# Autodesk Inventor assembly: HW2_1_task1_var4
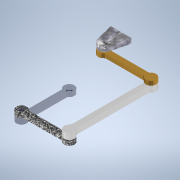
[picture p0: Inventor's stored thumbnail of the model, 180x180]
Saved by Autodesk Inventor 2022 (Build 260153000, 153)
## iProperties
Created: 2022-01-27
Part Number: HW2_1_task1_var4
Document SubType Name: Assembly
Designer: Administrator
Title: HW2_1_task1_var4 v1
Author: Administrator
## Documents named in this file (5)
- C:\Users\br4ch\M-and-Ms\HW2\Task3\Inventor\HW2_1_task1_var4.iam
- C:\Users\br4ch\M-and-Ms\HW2\Task3\Inventor\Machovik_Dlinn.ipt
- C:\Users\br4ch\M-and-Ms\HW2\Task3\Inventor\machovik_2_durki.ipt
- C:\Users\br4ch\M-and-Ms\HW2\Task3\Inventor\machovik.ipt
- C:\Users\br4ch\M-and-Ms\HW2\Task3\Inventor\kronsht.ipt
## Components (5 placed, 4 different names)
1. Machovik_Dlinn:1 — Cylindrical:2, Mate:2, Cylindrical:3, Mate:3, Angle:2, Angle:3
2. machovik_2_durki:1 — Cylindrical:3, Mate:3, Cylindrical:4, Mate:4, Angle:3, Angle:4
3. machovik:1 — Cylindrical:1, Mate:1, Cylindrical:2, Mate:2, Angle:1, Angle:2
4. kronsht:1 — Cylindrical:1, Mate:1, Angle:1
5. machovik:2 — Cylindrical:4, Mate:4, Angle:4
## Relationships (12: CylindricalJoint 4, Mate 4, Angle 4)
- Cylindrical:1: machovik:1 ↔ kronsht:1
- Mate:1 (3 mm): machovik:1 ↔ kronsht:1
- Cylindrical:2: Machovik_Dlinn:1 ↔ machovik:1
- Mate:2: Machovik_Dlinn:1 ↔ machovik:1
- Cylindrical:3: Machovik_Dlinn:1 ↔ machovik_2_durki:1
- Mate:3 (3 mm): Machovik_Dlinn:1 ↔ machovik_2_durki:1
- Cylindrical:4: machovik_2_durki:1 ↔ machovik:2
- Mate:4 (4 mm): machovik_2_durki:1 ↔ machovik:2
- Angle:1 (90 deg): machovik:1 ↔ kronsht:1
- Angle:2 (90 deg): Machovik_Dlinn:1 ↔ machovik:1
- Angle:3 (-90 deg): Machovik_Dlinn:1 ↔ machovik_2_durki:1
- Angle:4 (-90 deg): machovik_2_durki:1 ↔ machovik:2
